# Autodesk Inventor assembly: poleStandHorizAssyB
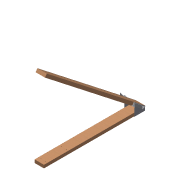
[picture p0: Inventor's stored thumbnail of the model, 180x180]
Saved by Autodesk Inventor 2017 (Build 210142000, 142)
## iProperties
Created: 2014-08-25
Part Number: poleStandHorizAssyB
Document SubType Name: Assembly
Designer: Dave
Author: Dave
## Documents named in this file (6)
- C:\Users\Kathryn Rosie\Google Drive\HERA\hera-cad-0\support\pole\poleStandHorizAssy.iam
- C:\Users\Kathryn Rosie\Google Drive\HERA\hera-cad-0\support\pole\poleStandHoriz2.ipt
- C:\Users\Kathryn Rosie\Google Drive\HERA\hera-cad-0\support\pole\poleStand37.ipt
- C:\Users\Kathryn Rosie\Google Drive\HERA\hera-cad-0\support\endcaps\Left\endcapLeft.iam
- endCapOptionLeft.iam
- C:\Users\Kathryn Rosie\Google Drive\HERA\hera-cad-0\support\endcaps\Right\endCapOptionRight.iam
## Components (4 placed, 4 different names)
1. endCapOptionLeft:1 [sub-assembly] — Mate:16, Mate:17, Flush:7, Mate:18, Mate:19, Mate:20, Flush:8
2. poleStandHoriz2:1 — Mate:16, Mate:17, Mate:20, Mate:21, Mate:22
3. poleStand37:1 — Flush:7, Mate:18, Mate:19
4. endCapOptionRight:1 [sub-assembly] — Mate:21, Mate:22, Flush:8
## Relationships (9: Mate 7, Flush 2)
- Mate:16: endCapOptionLeft:1 ↔ poleStandHoriz2:1
- Mate:17: endCapOptionLeft:1 ↔ poleStandHoriz2:1
- Flush:7: endCapOptionLeft:1 ↔ poleStand37:1
- Mate:18: endCapOptionLeft:1 ↔ poleStand37:1
- Mate:19: endCapOptionLeft:1 ↔ poleStand37:1
- Mate:20 (5.08 mm): endCapOptionLeft:1 ↔ poleStandHoriz2:1
- Mate:21: poleStandHoriz2:1 ↔ endCapOptionRight:1
- Mate:22: poleStandHoriz2:1 ↔ endCapOptionRight:1
- Flush:8: endCapOptionLeft:1 ↔ endCapOptionRight:1
